# Autodesk Inventor assembly: ASY ANP 1427 FDS way 7
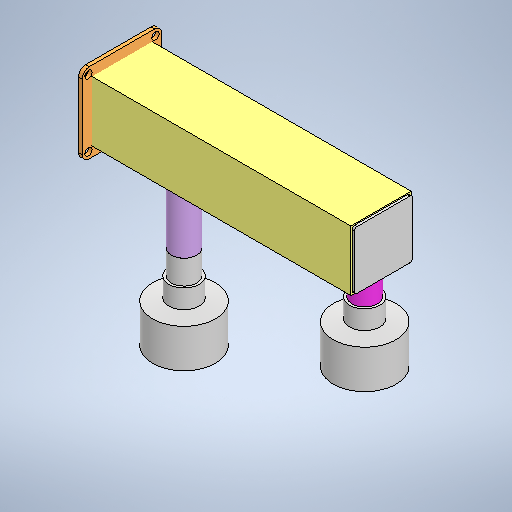
[picture p0: Inventor's stored thumbnail of the model, 512x512]
Saved by Autodesk Inventor 2025 (Build 290162010, 162A)
## iProperties
Created: 2025-07-02
Part Number: ASY ANP 1427 FDS way 7
Document SubType Name: Assembly
Designer: admin
Author: user
## Documents named in this file (7)
- C:\Users\admin\Yandex.Disk\home pc\Inventor\ANP--Antipayuta\FDS 1400\ASY ANP 1427 FDS way 7.iam
- C:\Users\admin\Yandex.Disk\home pc\Inventor\ANP--Antipayuta\FDS 1400\ANP 1437 FDS WAY tube7.ipt
- C:\Users\admin\Yandex.Disk\home pc\Inventor\ANP--Antipayuta\FDS 1400\ANP 1425 FDS Way FLANGE.ipt
- C:\Users\admin\Yandex.Disk\home pc\Inventor\ANP--Antipayuta\FDS 1400\ANP 1426 FDS way cup.ipt
- C:\Users\admin\Yandex.Disk\home pc\Inventor\ANP--Antipayuta\FDS 1400\ANP dummy filter element.ipt
- C:\Users\admin\Yandex.Disk\home pc\Inventor\ANP--Antipayuta\FDS 1400\ANP dummy pipe nippel.ipt
- C:\Users\admin\Yandex.Disk\home pc\Inventor\ANP--Antipayuta\FDS 1400\ANP 1451 FDS thread  tube10.ipt
## Components (8 placed, 6 different names)
1. ANP 1437 FDS WAY tube7.ipt:1 — Rigid:34, Rigid:35, Rigid:36, Rigid:27
2. ANP 1425 FDS Way FLANGE.ipt:1 — Rigid:34
3. ANP 1426 FDS way cup.ipt:1 — Rigid:35
4. ANP dummy filter element.ipt:2 — Rigid:33
5. ANP dummy pipe nippel.ipt:2 — Rigid:33, Rigid:36
6. ANP dummy filter element.ipt:5
7. ANP dummy pipe nippel.ipt:5
8. ANP 1451 FDS thread  tube10.ipt:3 — Rigid:27
## Relationships (7: WeldJoint 7)
- Rigid:34 [WeldJoint] (2 mm): ANP 1437 FDS WAY tube7.ipt:1 ↔ ANP 1425 FDS Way FLANGE.ipt:1
- Rigid:35 [WeldJoint]: ANP 1437 FDS WAY tube7.ipt:1 ↔ ANP 1426 FDS way cup.ipt:1
- Rigid:33 [WeldJoint]: ANP dummy filter element.ipt:2 ↔ ANP dummy pipe nippel.ipt:2
- Rigid:36 [WeldJoint]: ANP 1437 FDS WAY tube7.ipt:1 ↔ ANP dummy pipe nippel.ipt:2
- [WeldJoint]: ANP dummy filter element.ipt:5 ↔ ANP dummy pipe nippel.ipt:5
- [WeldJoint]: ANP dummy pipe nippel.ipt:5 ↔ ANP 1451 FDS thread  tube10.ipt:3
- Rigid:27 [WeldJoint]: ANP 1437 FDS WAY tube7.ipt:1 ↔ ANP 1451 FDS thread  tube10.ipt:3
## Named parameters: d24_d19 = 0 mm, d25_d21 = 0 mm
